# Autodesk Inventor assembly: 总装配
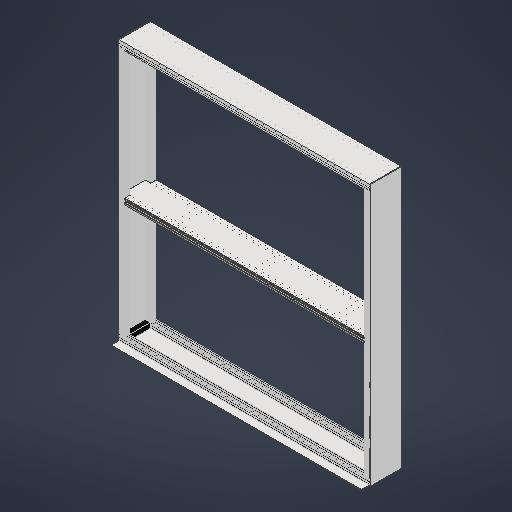
[picture p0: Inventor's stored thumbnail of the model, 512x512]
Saved by Autodesk Inventor 2025 (Build 290162000, 162)
## iProperties
Created: 2025-06-18
Part Number: 总装配
Document SubType Name: Assembly
Designer: XH
Author: XH
## Documents named in this file (10)
- C:\1A_Engineering_files\大众ID\总装配.iam
- C:\1A_Engineering_files\大众ID\零件1.ipt
- C:\1A_Engineering_files\大众ID\框架.ipt
- C:\1A_Engineering_files\大众ID\铝方管2020x.ipt
- C:\1A_Engineering_files\大众ID\板材.ipt
- C:\1A_Engineering_files\大众ID\板材2.ipt
- C:\1A_Engineering_files\大众ID\铝方管2020x60.ipt
- C:\1A_Engineering_files\大众ID\内板.ipt
- C:\1A_Engineering_files\大众ID\板材后.ipt
- C:\1A_Engineering_files\大众ID\铝方管2020中.ipt
## Components (26 placed, 9 different names)
1. 零件1:1 — 表面齐平:3, 表面齐平:14
2. 铝方管2020中:1 — 配合:33, 表面齐平:33, 表面齐平:34, 配合:35, 表面齐平:36, 配合:37, 配合:38, 表面齐平:40, 配合:39, 表面齐平:41
3. 铝方管2020中:2 — 表面齐平:34, 配合:34, 表面齐平:35, 表面齐平:38, 表面齐平:39
4. 铝方管2020x60:5 — 配合:35, 表面齐平:36
5. 铝方管2020x60:6 — 配合:36, 表面齐平:37, 表面齐平:38
6. 铝方管2020x60:7 — 配合:37, 表面齐平:39
7. 铝方管2020x60:8 — 配合:38, 表面齐平:40
8. 内板:3 — 配合:39, 表面齐平:41
9. 板材后:1 — 配合:31, 配合:32, 表面齐平:32
10. 内板:1 — 配合:28, 表面齐平:30
11. 内板:2 — 配合:30, 表面齐平:31
12. 板材:1 — 配合:6, 表面齐平:15, 表面齐平:17, 配合:9, 表面齐平:18, 表面齐平:19, 配合:17, 配合:20, 表面齐平:32
13. 板材:2 — 配合:7, 表面齐平:16, 表面齐平:17, 表面齐平:20, 配合:15, 配合:23, 配合:26, 配合:32
14. 板材2:1 — 配合:8, 配合:9, 表面齐平:18, 表面齐平:19, 表面齐平:20, 配合:14, 配合:16, 配合:25, 表面齐平:29
15. 框架:1 — 表面齐平:3, 表面齐平:4, 表面齐平:5, 表面齐平:7, 表面齐平:10, 配合:4, 配合:5, 表面齐平:12, 表面齐平:13, 配合:6, 表面齐平:15
16. 框架:2 — 表面齐平:4, 表面齐平:5, 表面齐平:11, 配合:7, 表面齐平:16, 表面齐平:35, 表面齐平:37
17. 铝方管2020x:1 — 表面齐平:7, 表面齐平:10, 配合:4, 表面齐平:11
18. 铝方管2020x:2 — 配合:5, 表面齐平:12, 表面齐平:13, 表面齐平:14, 配合:8
19. 铝方管2020x:3 — 配合:21, 配合:24, 配合:30, 表面齐平:31, 配合:31
20. 铝方管2020x:4 — 配合:14, 配合:18, 配合:27, 表面齐平:29, 配合:28, 表面齐平:30
21. 框架:3
22. 框架:4 — 配合:15, 配合:33, 表面齐平:33, 配合:34, 配合:36
23. 铝方管2020x60:1 — 配合:16, 配合:17, 配合:18
24. 铝方管2020x60:2 — 配合:20, 配合:21
25. 铝方管2020x60:3 — 配合:23, 配合:24
26. 铝方管2020x60:4 — 配合:25, 配合:26, 配合:27
## Relationships (66: Flush 35, Mate 31)
- 表面齐平:3 [Flush]: 零件1:1 ↔ 框架:1
- 表面齐平:4 [Flush]: 框架:1 ↔ 框架:2
- 表面齐平:5 [Flush]: 框架:1 ↔ 框架:2
- 表面齐平:7 [Flush]: 框架:1 ↔ 铝方管2020x:1
- 表面齐平:10 [Flush]: 框架:1 ↔ 铝方管2020x:1
- 配合:4 [Mate]: 框架:1 ↔ 铝方管2020x:1
- 表面齐平:11 [Flush]: 框架:2 ↔ 铝方管2020x:1
- 配合:5 [Mate]: 框架:1 ↔ 铝方管2020x:2
- 表面齐平:12 [Flush]: 框架:1 ↔ 铝方管2020x:2
- 表面齐平:13 [Flush]: 框架:1 ↔ 铝方管2020x:2
- 表面齐平:14 [Flush]: 零件1:1 ↔ 铝方管2020x:2
- 配合:6 [Mate]: 板材:1 ↔ 框架:1
- 表面齐平:15 [Flush]: 板材:1 ↔ 框架:1
- 配合:7 [Mate]: 板材:2 ↔ 框架:2
- 表面齐平:16 [Flush]: 板材:2 ↔ 框架:2
- 表面齐平:17 [Flush]: 板材:1 ↔ 板材:2
- 配合:8 [Mate]: 板材2:1 ↔ 铝方管2020x:2
- 配合:9 [Mate]: 板材:1 ↔ 板材2:1
- 表面齐平:18 [Flush]: 板材:1 ↔ 板材2:1
- 表面齐平:19 [Flush]: 板材:1 ↔ 板材2:1
- 表面齐平:20 [Flush]: 板材:2 ↔ 板材2:1
- [Flush]: 框架:3 ↔ 框架:4
- [Flush]: 框架:3 ↔ 框架:4
- [Flush]: 铝方管2020x:3 ↔ 框架:3
- [Flush]: 铝方管2020x:3 ↔ 框架:3
- [Mate]: 铝方管2020x:3 ↔ 框架:3
- [Flush]: 铝方管2020x:3 ↔ 框架:4
- [Mate]: 铝方管2020x:4 ↔ 框架:3
- [Flush]: 铝方管2020x:4 ↔ 框架:3
- [Flush]: 铝方管2020x:4 ↔ 框架:3
- 配合:14 [Mate]: 板材2:1 ↔ 铝方管2020x:4
- 配合:15 [Mate]: 板材:2 ↔ 框架:4
- 配合:16 [Mate]: 板材2:1 ↔ 铝方管2020x60:1
- 配合:17 [Mate]: 板材:1 ↔ 铝方管2020x60:1
- 配合:18 [Mate]: 铝方管2020x:4 ↔ 铝方管2020x60:1
- 配合:20 [Mate]: 板材:1 ↔ 铝方管2020x60:2
- 配合:21 [Mate]: 铝方管2020x:3 ↔ 铝方管2020x60:2
- 配合:23 [Mate]: 板材:2 ↔ 铝方管2020x60:3
- 配合:24 [Mate]: 铝方管2020x:3 ↔ 铝方管2020x60:3
- 配合:25 [Mate]: 板材2:1 ↔ 铝方管2020x60:4
- 配合:26 [Mate]: 板材:2 ↔ 铝方管2020x60:4
- 配合:27 [Mate]: 铝方管2020x:4 ↔ 铝方管2020x60:4
- 表面齐平:29 [Flush]: 板材2:1 ↔ 铝方管2020x:4
- 配合:28 [Mate]: 内板:1 ↔ 铝方管2020x:4
- 表面齐平:30 [Flush]: 内板:1 ↔ 铝方管2020x:4
- 配合:30 [Mate]: 内板:2 ↔ 铝方管2020x:3
- 表面齐平:31 [Flush]: 内板:2 ↔ 铝方管2020x:3
- 配合:31 [Mate]: 板材后:1 ↔ 铝方管2020x:3
- 配合:32 [Mate]: 板材后:1 ↔ 板材:2
- 表面齐平:32 [Flush]: 板材后:1 ↔ 板材:1
- 配合:33 [Mate]: 铝方管2020中:1 ↔ 框架:4
- 表面齐平:33 [Flush]: 铝方管2020中:1 ↔ 框架:4
- 表面齐平:34 [Flush]: 铝方管2020中:1 ↔ 铝方管2020中:2
- 配合:34 [Mate]: 铝方管2020中:2 ↔ 框架:4
- 表面齐平:35 [Flush]: 铝方管2020中:2 ↔ 框架:2
- 配合:35 [Mate]: 铝方管2020中:1 ↔ 铝方管2020x60:5
- 表面齐平:36 [Flush]: 铝方管2020中:1 ↔ 铝方管2020x60:5
- 配合:36 [Mate]: 铝方管2020x60:6 ↔ 框架:4
- 表面齐平:37 [Flush]: 铝方管2020x60:6 ↔ 框架:2
- 表面齐平:38 [Flush]: 铝方管2020中:2 ↔ 铝方管2020x60:6
- 配合:37 [Mate]: 铝方管2020中:1 ↔ 铝方管2020x60:7
- 表面齐平:39 [Flush]: 铝方管2020中:2 ↔ 铝方管2020x60:7
- 配合:38 [Mate]: 铝方管2020中:1 ↔ 铝方管2020x60:8
- 表面齐平:40 [Flush]: 铝方管2020中:1 ↔ 铝方管2020x60:8
- 配合:39 [Mate]: 铝方管2020中:1 ↔ 内板:3
- 表面齐平:41 [Flush]: 铝方管2020中:1 ↔ 内板:3
## Named parameters: d33_d3 = 0 mm, d34_d4 = 0 mm, d35_d8 = 0 mm, d36_d12 = 0 mm, d37_d13 = 0 mm, d38_d14 = 0 mm, d39_d15 = 0 mm, d40_d16 = 0 mm, d41_d17 = 0 mm
